# Autodesk Inventor assembly: Assembly1
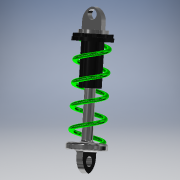
[picture p0: Inventor's stored thumbnail of the model, 180x180]
Saved by Autodesk Inventor 2019 (Build 230136000, 136)
## iProperties
Created: 2021-05-14
Part Number: Assembly1
Document SubType Name: Assembly
Designer: HP
Author: HP
## Documents named in this file (5)
- E:\Files and Documents\docs\Class Documents\Mechatronics\SES\Mechanical Design of Systems\Shock Breaker\Assembly1.iam
- E:\Files and Documents\docs\Class Documents\Mechatronics\SES\Mechanical Design of Systems\Shock Breaker\Part1.ipt
- E:\Files and Documents\docs\Class Documents\Mechatronics\SES\Mechanical Design of Systems\Shock Breaker\Part2.ipt
- E:\Files and Documents\docs\Class Documents\Mechatronics\SES\Mechanical Design of Systems\Shock Breaker\Part3.ipt
- E:\Files and Documents\docs\Class Documents\Mechatronics\SES\Mechanical Design of Systems\Shock Breaker\Part4.ipt
## Components (4 placed, 4 different names)
1. Part1:1 — Mate:1, Mate:2
2. Part2:1 — Mate:1, Mate:2, Mate:3, Mate:4, Mate:5
3. Part3:1 — Mate:3, Mate:4, Mate:6
4. Part4:1 — Mate:5, Mate:6
## Relationships (6: Mate 6)
- Mate:1: Part1:1 ↔ Part2:1
- Mate:2: Part1:1 ↔ Part2:1
- Mate:3: Part2:1 ↔ Part3:1
- Mate:4: Part2:1 ↔ Part3:1
- Mate:5: Part2:1 ↔ Part4:1
- Mate:6: Part3:1 ↔ Part4:1
